# Autodesk Inventor assembly: SplineAssembly
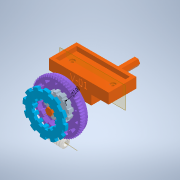
[picture p0: Inventor's stored thumbnail of the model, 180x180]
Saved by Autodesk Inventor 2021.2 (Build 252289000, 289)
## iProperties
Created: 2020-11-07
Part Number: SplineAssembly
Document SubType Name: Assembly
Designer: robst
Author: robst
## Documents named in this file (6)
- C:\git\CAD-Development\robSteele\ShapeWays\TelescopeProjects\TelescopeMount\SplineLock\SplineAssembly.iam
- C:\git\CAD-Development\robSteele\ShapeWays\TelescopeProjects\TelescopeMount\SplineLock\centerPartOfLock.ipt
- C:\git\CAD-Development\robSteele\ShapeWays\TelescopeProjects\TelescopeMount\SplineLock\outerPartOfLock.ipt
- C:\git\CAD-Development\robSteele\ShapeWays\TelescopeProjects\TelescopeMount\forkMountForDecTripV01\Design Accelerator\Worm Gears5.iam
- C:\git\CAD-Development\robSteele\ShapeWays\TelescopeProjects\TelescopeMount\hexBearing.ipt
- C:\git\CAD-Development\robSteele\ShapeWays\TelescopeProjects\TelescopeMount\connectorToTubeBracketWithOffsetHexShaft-V01.ipt
## Components (5 placed, 5 different names)
1. centerPartOfLock:1 — Insert:2
2. outerPartOfLock:1 — Insert:3, Mate:3
3. Worm Gears:1 [sub-assembly] — Insert:1, Insert:2, Insert:3, Mate:3
4. hexBearing:1 — Mate:1, Mate:2, Flush:1, Insert:1
5. connectorToTubeBracketWithOffsetHexShaft-V01:1 — Mate:1, Mate:2, Flush:1
## Relationships (7: Mate 3, Insert 3, Flush 1)
- Mate:1: hexBearing:1 ↔ connectorToTubeBracketWithOffsetHexShaft-V01:1
- Mate:2: hexBearing:1 ↔ connectorToTubeBracketWithOffsetHexShaft-V01:1
- Flush:1 (-25.4 mm): hexBearing:1 ↔ connectorToTubeBracketWithOffsetHexShaft-V01:1
- Insert:1: Worm Gears:1 ↔ hexBearing:1
- Insert:2: centerPartOfLock:1 ↔ Worm Gears:1
- Insert:3 (-25.4 mm): outerPartOfLock:1 ↔ Worm Gears:1
- Mate:3: outerPartOfLock:1 ↔ Worm Gears:1
